# Autodesk Inventor assembly: ダンパーアセンブリ_MIR1
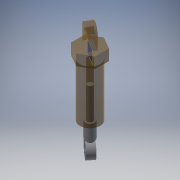
[picture p0: Inventor's stored thumbnail of the model, 180x180]
Saved by Autodesk Inventor 2016 (Build 200138000, 138)
## iProperties
Created: 2018-03-29
Part Number: ダンパーアセンブリ_MIR1
Material: 一般
Document SubType Name: Assembly
Designer: mozar
Mass: 15 g
Surface Area: 26.818 cm^2
Volume: 4.2661 cm^3
Density: 3.51609 g/cm^3
Author: Takumi
## Documents named in this file (3)
- C:\Users\mozar\Desktop\院2年機\既製品\ダンパーアセンブリ_MIR1.iam
- C:\Users\mozar\Desktop\院2年機\既製品\ダンパー下パーツ_MIR1.ipt
- C:\Users\mozar\Desktop\院2年機\既製品\ダンパー上パーツ_MIR1.ipt
## Components (2 placed, 2 different names)
1. ダンパー下パーツ_MIR1:1 — メイト:1
2. ダンパー上パーツ_MIR1:1 — メイト:1
## Relationships (1: Mate 1)
- メイト:1 [Mate]: ダンパー下パーツ_MIR1:1 ↔ ダンパー上パーツ_MIR1:1
